# Autodesk Inventor assembly: Ensamblaje_oso
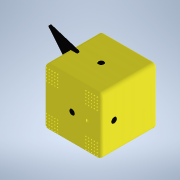
[picture p0: Inventor's stored thumbnail of the model, 180x180]
Saved by Autodesk Inventor 2021 (Build 250183000, 183)
## iProperties
Created: 2024-10-06
Part Number: Ensamblaje_oso
Document SubType Name: Assembly
Designer: hojan
Author: hojan
## Documents named in this file (8)
- C:\Users\hojan\Dropbox\Trabajos Personales\Nasa\Ensamblaje_oso.iam
- C:\Users\hojan\Dropbox\Trabajos Personales\Nasa\base_nasa.ipt
- C:\Users\hojan\Dropbox\Trabajos Personales\Nasa\cara_nasa.ipt
- C:\Users\hojan\Dropbox\Trabajos Personales\Nasa\gato.ipt
- C:\Users\hojan\Dropbox\Trabajos Personales\Nasa\pieza_nasa.ipt
- C:\Users\hojan\Dropbox\Trabajos Personales\Nasa\sensor.ipt
- C:\Users\hojan\Dropbox\Trabajos Personales\Nasa\sensor_2.ipt
- C:\Users\hojan\Dropbox\Trabajos Personales\Nasa\pantalla.ipt
## Components (13 placed, 7 different names)
1. base_nasa:1 — Coincidencia:1, Coincidencia:2, Coincidencia:3, Coincidencia:4, Coincidencia:5, Coincidencia:6, Coincidencia:7, Coincidencia:8, Coincidencia:9, Coincidencia:10, Coincidencia:15, Coincidencia:16, Coincidencia:17, Coincidencia:18, Coincidencia:19, Coincidencia:20, Coincidencia:26, Coincidencia:27, Coincidencia:28
2. cara_nasa:1 — Coincidencia:11, Coincidencia:12, Coincidencia:13, Coincidencia:14, Coincidencia:21, Coincidencia:22, Coincidencia:23, Coincidencia:24, Coincidencia:25, Nivelación:1, Coincidencia:26, Coincidencia:27, Coincidencia:28
3. gato:1 — Coincidencia:15, Coincidencia:16, Coincidencia:17
4. pieza_nasa:1 — Coincidencia:21, Coincidencia:22, Coincidencia:23
5. sensor:1 — Coincidencia:11, Coincidencia:12
6. sensor_2:1 — Coincidencia:1, Coincidencia:2
7. sensor_2:6 — Coincidencia:9, Coincidencia:10
8. sensor_2:8 — Coincidencia:3, Coincidencia:4
9. sensor_2:9 — Coincidencia:5, Coincidencia:6
10. sensor_2:10 — Coincidencia:7, Coincidencia:8
11. sensor:2 — Coincidencia:13, Coincidencia:14
12. gato:2 — Coincidencia:18, Coincidencia:19, Coincidencia:20
13. pantalla:1 — Coincidencia:24, Coincidencia:25, Nivelación:1
## Relationships (29: Mate 28, Flush 1)
- Coincidencia:1 [Mate]: base_nasa:1 ↔ sensor_2:1
- Coincidencia:2 [Mate]: base_nasa:1 ↔ sensor_2:1
- Coincidencia:3 [Mate]: base_nasa:1 ↔ sensor_2:8
- Coincidencia:4 [Mate]: base_nasa:1 ↔ sensor_2:8
- Coincidencia:5 [Mate]: base_nasa:1 ↔ sensor_2:9
- Coincidencia:6 [Mate]: base_nasa:1 ↔ sensor_2:9
- Coincidencia:7 [Mate]: base_nasa:1 ↔ sensor_2:10
- Coincidencia:8 [Mate]: base_nasa:1 ↔ sensor_2:10
- Coincidencia:9 [Mate]: base_nasa:1 ↔ sensor_2:6
- Coincidencia:10 [Mate]: base_nasa:1 ↔ sensor_2:6
- Coincidencia:11 [Mate]: cara_nasa:1 ↔ sensor:1
- Coincidencia:12 [Mate]: cara_nasa:1 ↔ sensor:1
- Coincidencia:13 [Mate]: cara_nasa:1 ↔ sensor:2
- Coincidencia:14 [Mate]: cara_nasa:1 ↔ sensor:2
- Coincidencia:15 [Mate]: base_nasa:1 ↔ gato:1
- Coincidencia:16 [Mate]: base_nasa:1 ↔ gato:1
- Coincidencia:17 [Mate]: base_nasa:1 ↔ gato:1
- Coincidencia:18 [Mate]: base_nasa:1 ↔ gato:2
- Coincidencia:19 [Mate]: base_nasa:1 ↔ gato:2
- Coincidencia:20 [Mate]: base_nasa:1 ↔ gato:2
- Coincidencia:21 [Mate]: cara_nasa:1 ↔ pieza_nasa:1
- Coincidencia:22 [Mate]: cara_nasa:1 ↔ pieza_nasa:1
- Coincidencia:23 [Mate]: cara_nasa:1 ↔ pieza_nasa:1
- Coincidencia:24 [Mate]: cara_nasa:1 ↔ pantalla:1
- Coincidencia:25 [Mate]: cara_nasa:1 ↔ pantalla:1
- Nivelación:1 [Flush]: cara_nasa:1 ↔ pantalla:1
- Coincidencia:26 [Mate]: base_nasa:1 ↔ cara_nasa:1
- Coincidencia:27 [Mate]: base_nasa:1 ↔ cara_nasa:1
- Coincidencia:28 [Mate]: base_nasa:1 ↔ cara_nasa:1
